# Autodesk Inventor assembly: Racks
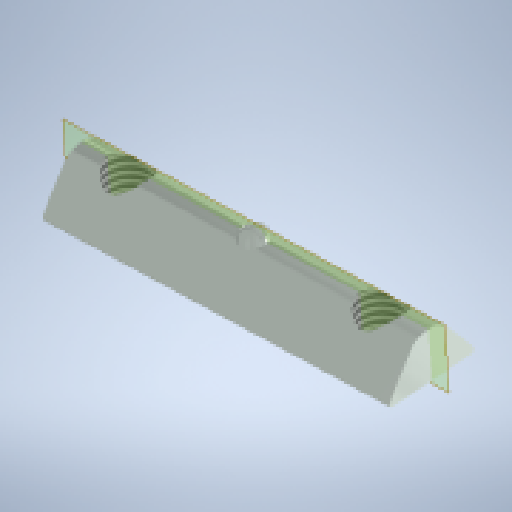
[picture p0: Inventor's stored thumbnail of the model, 512x512]
Saved by Autodesk Inventor 2023 (Build 270158000, 158)
## iProperties
Created: 2022-01-27
Part Number: Racks
Document SubType Name: Assembly
Designer: Elia
Author: Elia
## Documents named in this file (2)
- C:\Users\utente\OneDrive\Documenti\UniTN\I semestre\Mechanical Design\MDM-CyberOrto-CAD\Racks.iam
- C:\Users\utente\OneDrive\Documenti\UniTN\I semestre\Mechanical Design\MDM-CyberOrto-CAD\Parker components\02-Fasteners\10-Standard T-Nuts\20-050.ipt
## Components (1 placed, 1 different names)
1. 20-050:1 — Angolo:2, Allineato:3, Coincidente:5
## Relationships (4: Mate 2, Angle 1, Flush 1)
- Angolo:2 [Angle] (90 deg): 20-050:1
- Allineato:3 [Flush] (-27.5 mm): 20-050:1
- Coincidente:4 [Mate]
- Coincidente:5 [Mate]: 20-050:1
